# Autodesk Inventor assembly: Grid_Of_Piers
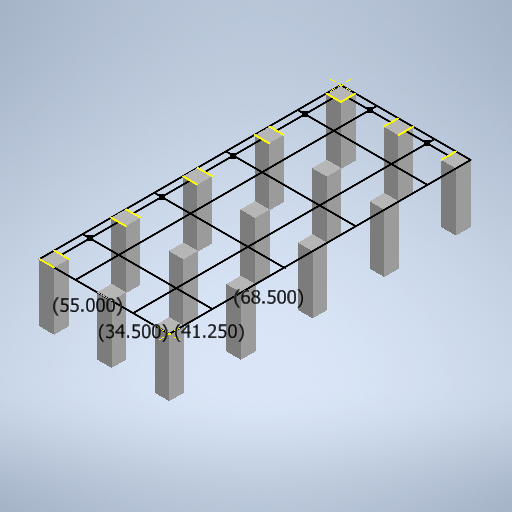
[picture p0: Inventor's stored thumbnail of the model, 512x512]
Saved by Autodesk Inventor 2025.1 (Build 291241020, 241B)
## iProperties
Created: 2024-08-07
Part Number: Grid_Of_Piers
Document SubType Name: Assembly
Designer: Tom
Author: Tom
## Documents named in this file (2)
- C:\Users\Tom\Documents\Inventor\Mobility\Additional_Building\Area_For_Additional_Buildings_With_Piers\Grid_Of_Piers.iam
- C:\Users\Tom\Documents\Inventor\Mobility\Additional_Building\Area_For_Additional_Buildings_With_Piers\Pier.ipt
## Components (15 placed, 1 different names)
1. Pier:1 — Mate:1, Mate:2, Mate:3
2. Pier:2
3. Pier:3
4. Pier:4
5. Pier:5
6. Pier:6
7. Pier:7
8. Pier:8
9. Pier:9
10. Pier:10
11. Pier:11
12. Pier:12
13. Pier:13
14. Pier:14
15. Pier:15
## Component patterns: (15 elements, first: Pier:1)
## Relationships (3: Mate 3)
- Mate:1: Pier:1
- Mate:2: Pier:1
- Mate:3: Pier:1
